# Autodesk Inventor assembly: cetakan sepatu
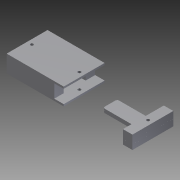
[picture p0: Inventor's stored thumbnail of the model, 180x180]
Saved by Autodesk Inventor 2012 (Build 160160000, 160)
## iProperties
Created: 2014-01-20
Part Number: cetakan sepatu
Document SubType Name: Assembly
Designer: Irwan Haryanto
Author: Irwan Haryanto
## Documents named in this file (6)
- D:\Renato\sepatu\cetakan sepatu.iam
- D:\Renato\sepatu\cetakan sepatu 1.ipt
- D:\Renato\sepatu\cetakan sepatu 2.ipt
- D:\Renato\sepatu\cetakan sepatu 3.ipt
- D:\Renato\sepatu\cetakan sepatu 4.ipt
- D:\Renato\sepatu\cetakan sepatu 5.ipt
## Components (10 placed, 5 different names)
1. cetakan sepatu 1:1 — Insert:1
2. cetakan sepatu 2:1 — Insert:2, Insert:3
3. cetakan sepatu 3:1 — Insert:1, Insert:2
4. cetakan sepatu 4:1 — Insert:6, Mate:1, Mate:2, Insert:7
5. cetakan sepatu 5:1 — Insert:6, Mate:1, Mate:2
6. cetakan sepatu 1:2 — Insert:5
7. cetakan sepatu 2:2 — Insert:3, Insert:4
8. cetakan sepatu 3:2 — Insert:4, Insert:5
9. cetakan sepatu 4:2 — Insert:7, Insert:8, Mate:3
10. cetakan sepatu 5:2 — Insert:8, Mate:3
## Relationships (11: Insert 8, Mate 3)
- Insert:1: cetakan sepatu 1:1 ↔ cetakan sepatu 3:1
- Insert:2: cetakan sepatu 2:1 ↔ cetakan sepatu 3:1
- Insert:3: cetakan sepatu 2:1 ↔ cetakan sepatu 2:2
- Insert:4: cetakan sepatu 2:2 ↔ cetakan sepatu 3:2
- Insert:5: cetakan sepatu 1:2 ↔ cetakan sepatu 3:2
- Insert:6: cetakan sepatu 4:1 ↔ cetakan sepatu 5:1
- Mate:1: cetakan sepatu 4:1 ↔ cetakan sepatu 5:1
- Mate:2: cetakan sepatu 4:1 ↔ cetakan sepatu 5:1
- Insert:7: cetakan sepatu 4:1 ↔ cetakan sepatu 4:2
- Insert:8: cetakan sepatu 4:2 ↔ cetakan sepatu 5:2
- Mate:3: cetakan sepatu 4:2 ↔ cetakan sepatu 5:2
